# Autodesk Inventor assembly: SA-R3
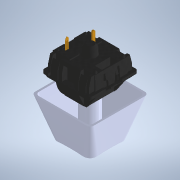
[picture p0: Inventor's stored thumbnail of the model, 180x180]
Saved by Autodesk Inventor 2020 (Build 240168000, 168)
## iProperties
Created: 2019-07-03
Part Number: SA-R3
Document SubType Name: Assembly
Designer: Thibault
Mass: 0.99122 g
Surface Area: 32.3296 cm^2
Volume: 0.99122 cm^3
Density: 1 g/cm^3
Sending System: Creo  TM  3.0
Author: Thibault
## Documents named in this file (28)
- C:\Users\Thibault Polge\Documents\Habilis\mech\mx.iam
- C:\Users\Thibault Polge\Documents\Habilis\mech\MX_DOWN.ipt
- C:\Users\Thibault Polge\Documents\Habilis\mech\MX_UP.ipt
- C:\Users\Thibault Polge\Documents\Habilis\mech\MX_PIN.ipt
- C:\Users\Thibault Polge\Documents\Habilis\mech\MX_SPRING.ipt
- C:\Users\Thibault Polge\Documents\Habilis\mech\MX_CLICK.ipt
- C:\Users\Thibault Polge\Documents\Habilis\mech\mx_stem.ipt
- C:\Users\Thibault Polge\Documents\Habilis\mech\keycaps\1x1 R1 v23.ipt
- C:\Users\Thibault Polge\Documents\Habilis\mech\keycaps\1x1 R2 v8.ipt
- C:\Users\Thibault Polge\Documents\Habilis\mech\keycaps\1x1 R3 v8.ipt
- C:\Users\Thibault Polge\Documents\Habilis\mech\keycaps\1x1 R4 v6.ipt
- C:\Users\Thibault Polge\Documents\Habilis\mech\keycaps\1x2 R1 v6.ipt
- C:\Users\Thibault Polge\Documents\Habilis\mech\mx_stem\Brown.ipt
- C:\Users\Thibault Polge\Documents\Habilis\mech\keycap_dsa_1x1.ipt
- C:\Users\Thibault Polge\Documents\Habilis\mech\keycap_sa_r3.ipt
- Blue-0.iam
- Brown-0.iam
- DSA-1x1.iam
- R1.iam
- R2.iam
- R3.iam
- R4.iam
- SA-R3.iam
- TC-R1.iam
- TC-R1 2×1 A.iam
- TC-R1 2×1 B.iam
- TC-R3.iam
- TC-R4.iam
## Components (13 placed, 13 different names)
1. MX_DOWN — Placage:1, Placage:2, Angle:1, Angle:3
2. MX_UP — Placage:3, Angle:2, Angle:4, Angle:5
3. UP_MX — Placage:1, Placage:2, Placage:3, Placage:4, Placage:5, Placage:6, Placage:7, Placage:8, Placage:9, Placage:10, Placage:11, Placage:12, Placage:13, Placage:14, Placage:15, Placage:16, Placage:17, Placage:18, Placage:19
4. MX_PIN
5. MX_SPRING
6. MX_CLICK
7. 1x1 R1 — Placage:4, Placage:5, Angle:1
8. 1x1 R2 — Placage:6, Angle:2, Placage:7
9. 1x1 R3 — Placage:8, Angle:3, Placage:9
10. 1x1 R4 — Placage:10, Angle:4, Placage:11
11. 1x2 R1 v6:1 — Placage:12, Angle:5, Placage:13
12. keycap_dsa_1x1:1 — Placage:14, Placage:15, Placage:16
13. keycap_sa_r3:1 — Placage:17, Placage:18, Placage:19
## Relationships (24: Mate 19, Angle 5)
- Placage:1 [Mate]: MX_DOWN ↔ UP_MX
- Placage:2 [Mate]: MX_DOWN ↔ UP_MX
- Placage:3 [Mate]: MX_UP ↔ UP_MX
- Placage:4 [Mate]: UP_MX ↔ 1x1 R1
- Placage:5 [Mate]: UP_MX ↔ 1x1 R1
- Angle:1 (0 deg): MX_DOWN ↔ 1x1 R1
- Placage:6 [Mate]: UP_MX ↔ 1x1 R2
- Angle:2 (0 deg): MX_UP ↔ 1x1 R2
- Placage:7 [Mate]: UP_MX ↔ 1x1 R2
- Placage:8 [Mate]: UP_MX ↔ 1x1 R3
- Angle:3 (90 deg): MX_DOWN ↔ 1x1 R3
- Placage:9 [Mate]: UP_MX ↔ 1x1 R3
- Placage:10 [Mate]: UP_MX ↔ 1x1 R4
- Angle:4 (90 deg): MX_UP ↔ 1x1 R4
- Placage:11 [Mate]: UP_MX ↔ 1x1 R4
- Placage:12 [Mate]: UP_MX ↔ 1x2 R1 v6:1
- Angle:5 (0 deg): MX_UP ↔ 1x2 R1 v6:1
- Placage:13 [Mate]: UP_MX ↔ 1x2 R1 v6:1
- Placage:14 [Mate]: UP_MX ↔ keycap_dsa_1x1:1
- Placage:15 [Mate]: UP_MX ↔ keycap_dsa_1x1:1
- Placage:16 [Mate]: UP_MX ↔ keycap_dsa_1x1:1
- Placage:17 [Mate]: UP_MX ↔ keycap_sa_r3:1
- Placage:18 [Mate]: UP_MX ↔ keycap_sa_r3:1
- Placage:19 [Mate]: UP_MX ↔ keycap_sa_r3:1
